# Autodesk Inventor assembly: Steel Ball Bearing (6383K245)
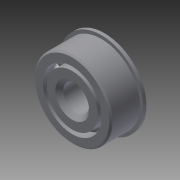
[picture p0: Inventor's stored thumbnail of the model, 180x180]
Saved by Autodesk Inventor 2015 (Build 190159000, 159)
## iProperties
Created: 2014-05-18
Part Number: Steel Ball Bearing (6383K245)
Document SubType Name: Assembly
Designer: seaha_000
Mass: 14.2123 g
Surface Area: 93.5025 cm^2
Volume: 14.2123 cm^3
Density: 1 g/cm^3
Author: seaha_000
## Documents named in this file (16)
- X:\Dropbox\_School\AimBot\Steel Ball Bearing (6383K245).iam
- X:\Dropbox\_School\AimBot\Imported Components\6383K245\Part45.ipt
- X:\Dropbox\_School\AimBot\Imported Components\6383K245\Part47.ipt
- X:\Dropbox\_School\AimBot\Imported Components\6383K245\Part49.ipt
- X:\Dropbox\_School\AimBot\Imported Components\6383K245\Part51.ipt
- X:\Dropbox\_School\AimBot\Imported Components\6383K245\Part53.ipt
- X:\Dropbox\_School\AimBot\Imported Components\6383K245\Part55.ipt
- X:\Dropbox\_School\AimBot\Imported Components\6383K245\Part57.ipt
- X:\Dropbox\_School\AimBot\Imported Components\6383K245\Part59.ipt
- X:\Dropbox\_School\AimBot\Imported Components\6383K245\Part61.ipt
- X:\Dropbox\_School\AimBot\Imported Components\6383K245\Part63.ipt
- X:\Dropbox\_School\AimBot\Imported Components\6383K245\Part65.ipt
- X:\Dropbox\_School\AimBot\Imported Components\6383K245\Part67.ipt
- X:\Dropbox\_School\AimBot\Imported Components\6383K245\Part69.ipt
- X:\Dropbox\_School\AimBot\Imported Components\6383K245\Part71.ipt
- X:\Dropbox\_School\AimBot\Imported Components\6383K245\Part73.ipt
## Components (15 placed, 15 different names)
1. Part45:1 — Cylindrical:1, Flush:1
2. Part47:1
3. Part49:1
4. Part51:1
5. Part53:1
6. Part55:1
7. Part57:1
8. Part59:1
9. Part61:1
10. Part63:1
11. Part65:1
12. Part67:1
13. Part69:1
14. Part71:1
15. Part73:1 — Cylindrical:1, Flush:1
## Relationships (2: CylindricalJoint 1, Flush 1)
- Cylindrical:1: Part45:1 ↔ Part73:1
- Flush:1: Part45:1 ↔ Part73:1
